# Autodesk Inventor assembly: Assembly-ASI-54-12-8
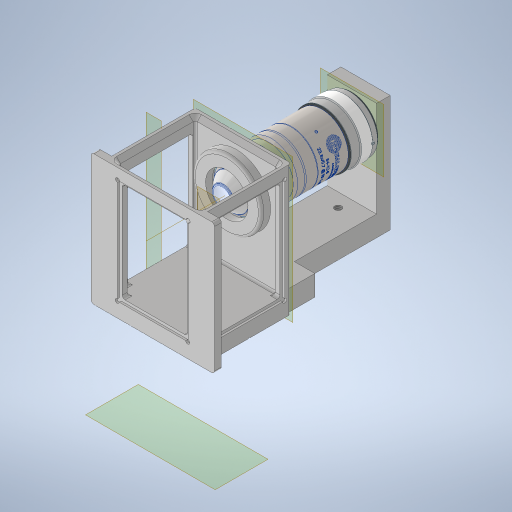
[picture p0: Inventor's stored thumbnail of the model, 512x512]
Saved by Autodesk Inventor 2024 (Build 280153000, 153)
## iProperties
Created: 2026-02-24
Part Number: Assembly-ASI-54-12-8
Document SubType Name: Assembly
Designer: nvladi
Author: nvladi
## Documents named in this file (5)
- C:\Users\nvladi\Documents\GitHub\benchtop-hardware\Benchtop-2024(default-version)\custom-parts\sample_handling\3Dprinted-immersion-chamber-Slides-50x75mm-ASI-immersion-objective\Assembly-ASI-54-12-8.iam
- C:\Users\nvladi\Documents\GitHub\benchtop-hardware\Benchtop-2024(default-version)\custom-parts\sample_handling\3Dprinted-immersion-chamber-Slides-50x75mm-ASI-immersion-objective\cuvette-w70mm-slide50x75mm-O-ringOD42mm.ipt
- C:\Users\nvladi\Documents\GitHub\benchtop-hardware\Benchtop-2024(default-version)\CAD-model-Inventor\library\ASI\54-12-8 REV A (CATALOG MODEL)\54-12-8 REV A (CATALOG MODEL).ipt
- C:\Users\nvladi\Documents\GitHub\benchtop-hardware\Benchtop-2024(default-version)\CAD-model-Inventor\library\Thorlabs\lens_tubes\SM1ZM.ipt
- C:\Users\nvladi\Documents\GitHub\benchtop-hardware\Benchtop-2024(default-version)\custom-parts\sample_handling\3Dprinted-immersion-chamber-Slides-50x75mm-ASI-immersion-objective\AdapterBracket.ipt
## Components (4 placed, 4 different names)
1. cuvette-w70mm-slide50x75mm-O-ringOD42mm:1 — Mate:1, Mate:2, Flush:2, Flush:3
2. 54-12-8 REV A (CATALOG MODEL):1 — Mate:1, Mate:3, Insert:1
3. SM1ZM:1 — Insert:1, Flush:1
4. AdapterBracket:1 — Flush:2, Flush:3
## Relationships (8: Mate 4, Flush 3, Insert 1)
- Mate:1: cuvette-w70mm-slide50x75mm-O-ringOD42mm:1 ↔ 54-12-8 REV A (CATALOG MODEL):1
- Mate:2: cuvette-w70mm-slide50x75mm-O-ringOD42mm:1
- Mate:3: 54-12-8 REV A (CATALOG MODEL):1
- Mate:4
- Insert:1: 54-12-8 REV A (CATALOG MODEL):1 ↔ SM1ZM:1
- Flush:1: SM1ZM:1
- Flush:2: cuvette-w70mm-slide50x75mm-O-ringOD42mm:1 ↔ AdapterBracket:1
- Flush:3: cuvette-w70mm-slide50x75mm-O-ringOD42mm:1 ↔ AdapterBracket:1
